# Autodesk Inventor assembly: 바퀴 서브 조립
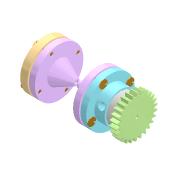
[picture p0: Inventor's stored thumbnail of the model, 180x180]
Saved by Autodesk Inventor 2020 (Build 240168000, 168)
## iProperties
Created: 2020-06-01
Part Number: 바퀴 서브 조립
Document SubType Name: Assembly
Designer: Miji
Author: Miji
## Documents named in this file (9)
- C:\Users\82102\OneDrive\바탕 화면\개인자료\졸업과제\설계\로봇\모델링 1.2\바퀴 서브 조립.iam
- C:\Users\82102\OneDrive\바탕 화면\개인자료\졸업과제\설계\로봇\모델링 1.2\메인 스퍼기어 부시.ipt
- C:\Users\82102\OneDrive\바탕 화면\개인자료\졸업과제\설계\로봇\모델링 1.2\메인 스퍼기어.ipt
- C:\Users\82102\OneDrive\바탕 화면\개인자료\졸업과제\설계\로봇\모델링 1.2\바퀴.ipt
- C:\Users\82102\OneDrive\바탕 화면\개인자료\졸업과제\설계\로봇\모델링 1.2\외부 바퀴 서포터.ipt
- C:\Users\82102\OneDrive\바탕 화면\개인자료\졸업과제\설계\로봇\모델링 1.2\메인 바퀴 간격링.ipt
- C:\Users\82102\OneDrive\바탕 화면\개인자료\졸업과제\설계\로봇\모델링 1.2\메인 바퀴 서포터.ipt
- C:\Users\82102\OneDrive\바탕 화면\개인자료\졸업과제\설계\로봇\모델링 1.2\규격품\볼트 3M 6L.ipt
- C:\Users\82102\OneDrive\바탕 화면\개인자료\졸업과제\설계\로봇\모델링 1.2\지름 니플.ipt
## Components (16 placed, 8 different names)
1. 메인 스퍼기어 부시:1 — 메이트:1, 메이트:2
2. 메인 스퍼기어:1 — 메이트:1, 메이트:2, 메이트:3, 메이트:4
3. 바퀴:1 — 메이트:5, 메이트:6, 메이트:7, 메이트:8, 메이트:10, 메이트:11, 메이트:12, 메이트:13, 메이트:14, 메이트:15, 메이트:16
4. 외부 바퀴 서포터:1 — 메이트:14, 메이트:15, 메이트:16, 메이트:22, 메이트:23, 메이트:24, 메이트:25, 메이트:26, 메이트:27, 메이트:28
5. 메인 바퀴 간격링:1 — 메이트:3, 메이트:4, 메이트:5, 메이트:9, 메이트:10, 메이트:17, 각도:1, 메이트:18, 메이트:19, 메이트:20, 메이트:21
6. 메인 바퀴 서포터:1 — 메이트:6, 메이트:7, 메이트:8, 메이트:9
7. 메인 바퀴 서포터:2 — 메이트:11, 메이트:12, 메이트:13
8. 볼트 3M 6L:1 — 메이트:17, 각도:1, 각도:2, 플러쉬:10, 메이트:21
9. 볼트 3M 6L:2 — 메이트:18, 각도:2, 각도:3, 플러쉬:10, 플러쉬:9
10. 볼트 3M 6L:3 — 메이트:20, 각도:3, 각도:4, 플러쉬:9, 플러쉬:8
11. 볼트 3M 6L:4 — 메이트:19, 각도:4, 플러쉬:8
12. 볼트 3M 6L:5 — 메이트:23
13. 볼트 3M 6L:6 — 메이트:25, 메이트:26
14. 볼트 3M 6L:7 — 메이트:24
15. 볼트 3M 6L:8 — 메이트:22
16. 지름 니플:1 — 메이트:27, 메이트:28
## Relationships (41: Mate 28, Angle 7, Flush 6)
- 메이트:1 [Mate]: 메인 스퍼기어 부시:1 ↔ 메인 스퍼기어:1
- 메이트:2 [Mate]: 메인 스퍼기어 부시:1 ↔ 메인 스퍼기어:1
- 메이트:3 [Mate]: 메인 스퍼기어:1 ↔ 메인 바퀴 간격링:1
- 메이트:4 [Mate]: 메인 스퍼기어:1 ↔ 메인 바퀴 간격링:1
- 메이트:5 [Mate]: 바퀴:1 ↔ 메인 바퀴 간격링:1
- 메이트:6 [Mate]: 바퀴:1 ↔ 메인 바퀴 서포터:1
- 메이트:7 [Mate]: 바퀴:1 ↔ 메인 바퀴 서포터:1
- 메이트:8 [Mate]: 바퀴:1 ↔ 메인 바퀴 서포터:1
- 메이트:9 [Mate]: 메인 바퀴 간격링:1 ↔ 메인 바퀴 서포터:1
- 메이트:10 [Mate]: 바퀴:1 ↔ 메인 바퀴 간격링:1
- 메이트:11 [Mate]: 바퀴:1 ↔ 메인 바퀴 서포터:2
- 메이트:12 [Mate]: 바퀴:1 ↔ 메인 바퀴 서포터:2
- 메이트:13 [Mate]: 바퀴:1 ↔ 메인 바퀴 서포터:2
- 메이트:14 [Mate]: 바퀴:1 ↔ 외부 바퀴 서포터:1
- 메이트:15 [Mate]: 바퀴:1 ↔ 외부 바퀴 서포터:1
- 메이트:16 [Mate]: 바퀴:1 ↔ 외부 바퀴 서포터:1
- 메이트:17 [Mate]: 메인 바퀴 간격링:1 ↔ 볼트 3M 6L:1
- 각도:1 [Angle] (0 deg): 메인 바퀴 간격링:1 ↔ 볼트 3M 6L:1
- 메이트:18 [Mate]: 메인 바퀴 간격링:1 ↔ 볼트 3M 6L:2
- 메이트:19 [Mate]: 메인 바퀴 간격링:1 ↔ 볼트 3M 6L:4
- 메이트:20 [Mate]: 메인 바퀴 간격링:1 ↔ 볼트 3M 6L:3
- 각도:2 [Angle] (0 deg): 볼트 3M 6L:1 ↔ 볼트 3M 6L:2
- 각도:3 [Angle] (0 deg): 볼트 3M 6L:2 ↔ 볼트 3M 6L:3
- 각도:4 [Angle] (0 deg): 볼트 3M 6L:3 ↔ 볼트 3M 6L:4
- 플러쉬:10 [Flush]: 볼트 3M 6L:1 ↔ 볼트 3M 6L:2
- 플러쉬:9 [Flush]: 볼트 3M 6L:2 ↔ 볼트 3M 6L:3
- 플러쉬:8 [Flush]: 볼트 3M 6L:3 ↔ 볼트 3M 6L:4
- 메이트:21 [Mate]: 메인 바퀴 간격링:1 ↔ 볼트 3M 6L:1
- [Angle] (0 deg): 볼트 3M 6L:5 ↔ 볼트 3M 6L:6
- [Angle] (0 deg): 볼트 3M 6L:6 ↔ 볼트 3M 6L:7
- [Angle] (0 deg): 볼트 3M 6L:7 ↔ 볼트 3M 6L:8
- [Flush]: 볼트 3M 6L:5 ↔ 볼트 3M 6L:6
- [Flush]: 볼트 3M 6L:6 ↔ 볼트 3M 6L:7
- [Flush]: 볼트 3M 6L:7 ↔ 볼트 3M 6L:8
- 메이트:22 [Mate]: 외부 바퀴 서포터:1 ↔ 볼트 3M 6L:8
- 메이트:23 [Mate]: 외부 바퀴 서포터:1 ↔ 볼트 3M 6L:5
- 메이트:24 [Mate]: 외부 바퀴 서포터:1 ↔ 볼트 3M 6L:7
- 메이트:25 [Mate]: 외부 바퀴 서포터:1 ↔ 볼트 3M 6L:6
- 메이트:26 [Mate]: 외부 바퀴 서포터:1 ↔ 볼트 3M 6L:6
- 메이트:27 [Mate]: 외부 바퀴 서포터:1 ↔ 지름 니플:1
- 메이트:28 [Mate]: 외부 바퀴 서포터:1 ↔ 지름 니플:1
## Named parameters: d31_d22 = 0 deg, d32_d23 = 0 deg, d33_d27 = 0 mm, d34_d21 = 0 deg, d35_d28 = 0 mm, d36_d29 = 0 mm
